# Autodesk Inventor assembly: CH3-chassisFull
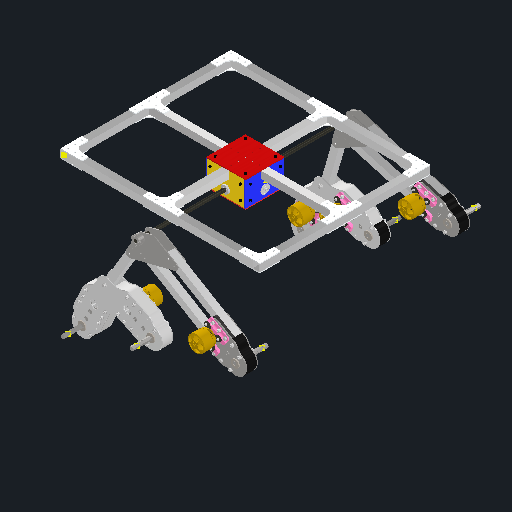
[picture p0: Inventor's stored thumbnail of the model, 512x512]
Saved by Autodesk Inventor 2026.1 (Build 301233020, 233B)
## iProperties
Created: 2025-01-30
Part Number: CH3-chassisFull
Document SubType Name: Assembly
Designer: t205b
Author: t205b
## Documents named in this file (15)
- C:\Users\t205b\OneDrive\Documents\Github\BehrendURCMechanical\CAD\Chassis V3\CH3-chassisFull.iam
- C:\Users\t205b\OneDrive\Documents\Github\BehrendURCMechanical\CAD\Chassis V3\aluminumextrusiontool.ipt
- C:\Users\t205b\OneDrive\Documents\Github\BehrendURCMechanical\CAD\Chassis V3\CH3-L3DoubleGearbox.iam
- C:\Users\t205b\OneDrive\Documents\Github\BehrendURCMechanical\CAD\Chassis V3\CH3-L1SingleGearbox.iam
- C:\Users\t205b\OneDrive\Documents\Github\BehrendURCMechanical\CAD\Chassis V3\HipPivotPlate.ipt
- C:\Users\t205b\OneDrive\Documents\Github\BehrendURCMechanical\CAD\Chassis V3\CH3-PivotBoltNutWasher.iam
- C:\Users\t205b\OneDrive\Documents\Github\BehrendURCMechanical\CAD\Chassis V3\aluminumextrusiontool\aluminumextrusiontool-13.31255in.ipt
- C:\Users\t205b\OneDrive\Documents\Github\BehrendURCMechanical\CAD\Chassis V3\aluminumextrusiontool\aluminumextrusiontool\aluminumextrusiontool-17-13.31255in.ipt
- C:\Users\t205b\OneDrive\Documents\Github\BehrendURCMechanical\CAD\Chassis V3\aluminumextrusiontool\aluminumextrusiontool.ipt
- C:\Users\t205b\OneDrive\Documents\Github\BehrendURCMechanical\CAD\Chassis V3\aluminumextrusiontool\aluminumextrusiontool\aluminumextrusiontool-8in.ipt
- C:\Users\t205b\OneDrive\Documents\Github\BehrendURCMechanical\CAD\Chassis V3\aluminumextrusiontool\aluminumextrusiontool\aluminumextrusiontool-11in.ipt
- C:\Users\t205b\OneDrive\Documents\Github\BehrendURCMechanical\CAD\Chassis V3\Body\CH3-BodyAssembly.iam
- C:\Users\t205b\OneDrive\Documents\Github\BehrendURCMechanical\CAD\Chassis V3\Differential Box\CH3-DiffHousingAsm.iam
- C:\Users\t205b\OneDrive\Documents\Github\BehrendURCMechanical\CAD\Chassis V3\HipCoupler.ipt
- C:\Users\t205b\OneDrive\Documents\Github\BehrendURCMechanical\CAD\Chassis V3\HipCoupler V2.ipt
## Components (22 placed, 12 different names)
1. aluminumextrusiontool-17-13.5in:11 — Mate:31, Mate:32, Mate:33, Mate:38
2. aluminumextrusiontool-8in:12 — Mate:9, Mate:10, Mate:15, Mate:16, Mate:17, Mate:18, Mate:19, Mate:20
3. CH3-L3DoubleGearbox:1 [sub-assembly] — Mate:29, Mate:30
4. CH3-L3DoubleGearbox:2 [sub-assembly] — Mate:4, Mate:5, Mate:22
5. CH3-L1SingleGearbox:1 [sub-assembly] — Mate:37, Mate:38, Mate:39
6. CH3-L1SingleGearbox:2 [sub-assembly] — Mate:46, Mate:47, Mate:48
7. HipPivotPlate:1 — Mate:10, Mate:19, Mate:20, Mate:54, Mate:58, Mate:60
8. HipPivotPlate:2 — Mate:26, Mate:27, Mate:28, Mate:40, Mate:41, Mate:43, Mate:44, Mate:62, Mate:63
9. CH3-PivotBoltNutWasher:1 [sub-assembly] — Mate:9, Mate:16, Mate:29, Mate:30
10. CH3-PivotBoltNutWasher:2 [sub-assembly] — Mate:4, Mate:5, Mate:21
11. HipPivotPlate:3 — Mate:15, Mate:17, Mate:18, Mate:31, Mate:32, Mate:33, Mate:34, Mate:35, Mate:36, Mate:56, Mate:57
12. aluminumextrusiontool-11in:13 — Mate:43, Mate:44, Mate:45, Mate:46
13. aluminumextrusiontool-11in:14 — Mate:34, Mate:35, Mate:36, Mate:37, Mate:39
14. aluminumextrusiontool-13.31255in:10 — Mate:40, Mate:41, Mate:42, Mate:47, Mate:48
15. aluminumextrusiontool-8in:15 — Mate:21, Mate:22, Mate:23, Mate:24, Mate:25, Mate:26, Mate:27, Mate:28
16. HipPivotPlate:4 — Mate:23, Mate:24, Mate:25, Mate:42, Mate:45, Mate:53, Mate:64, Mate:65, Mate:66
17. CH3-BodyAssembly:1 [sub-assembly] — Mate:49, Mate:50, Mate:51, Mate:52
18. Ch3-DiffHousingAsm:1 [sub-assembly] — Mate:49, Mate:50, Mate:51, Mate:52, Mate:53, Mate:54, Mate:55, Mate:59, Mate:61, Flush:1, Flush:2
19. HipCoupler:1 — Mate:58, Mate:59, Mate:60
20. HipCoupler V2:1 — Mate:55, Mate:56, Mate:57, Flush:1
21. HipCoupler:2 — Mate:61, Mate:62, Mate:63
22. HipCoupler V2:2 — Mate:64, Mate:65, Mate:66, Flush:2
## Relationships (58: Mate 56, Flush 2)
- Mate:4: CH3-L3DoubleGearbox:2 ↔ CH3-PivotBoltNutWasher:2
- Mate:5: CH3-L3DoubleGearbox:2 ↔ CH3-PivotBoltNutWasher:2
- Mate:9: aluminumextrusiontool-8in:12 ↔ CH3-PivotBoltNutWasher:1
- Mate:10: aluminumextrusiontool-8in:12 ↔ HipPivotPlate:1
- Mate:15: aluminumextrusiontool-8in:12 ↔ HipPivotPlate:3
- Mate:16: aluminumextrusiontool-8in:12 ↔ CH3-PivotBoltNutWasher:1
- Mate:17: aluminumextrusiontool-8in:12 ↔ HipPivotPlate:3
- Mate:18: aluminumextrusiontool-8in:12 ↔ HipPivotPlate:3
- Mate:19: aluminumextrusiontool-8in:12 ↔ HipPivotPlate:1
- Mate:20: aluminumextrusiontool-8in:12 ↔ HipPivotPlate:1
- Mate:21: CH3-PivotBoltNutWasher:2 ↔ aluminumextrusiontool-8in:15
- Mate:22: CH3-L3DoubleGearbox:2 ↔ aluminumextrusiontool-8in:15
- Mate:23: aluminumextrusiontool-8in:15 ↔ HipPivotPlate:4
- Mate:24: aluminumextrusiontool-8in:15 ↔ HipPivotPlate:4
- Mate:25: aluminumextrusiontool-8in:15 ↔ HipPivotPlate:4
- Mate:26: HipPivotPlate:2 ↔ aluminumextrusiontool-8in:15
- Mate:27: HipPivotPlate:2 ↔ aluminumextrusiontool-8in:15
- Mate:28: HipPivotPlate:2 ↔ aluminumextrusiontool-8in:15
- Mate:29: CH3-L3DoubleGearbox:1 ↔ CH3-PivotBoltNutWasher:1
- Mate:30: CH3-L3DoubleGearbox:1 ↔ CH3-PivotBoltNutWasher:1
- Mate:31: aluminumextrusiontool-17-13.5in:11 ↔ HipPivotPlate:3
- Mate:32: aluminumextrusiontool-17-13.5in:11 ↔ HipPivotPlate:3
- Mate:33: aluminumextrusiontool-17-13.5in:11 ↔ HipPivotPlate:3
- Mate:34: HipPivotPlate:3 ↔ aluminumextrusiontool-11in:14
- Mate:35: HipPivotPlate:3 ↔ aluminumextrusiontool-11in:14
- Mate:36: HipPivotPlate:3 ↔ aluminumextrusiontool-11in:14
- Mate:37: CH3-L1SingleGearbox:1 ↔ aluminumextrusiontool-11in:14
- Mate:38: aluminumextrusiontool-17-13.5in:11 ↔ CH3-L1SingleGearbox:1
- Mate:39: CH3-L1SingleGearbox:1 ↔ aluminumextrusiontool-11in:14
- Mate:40: HipPivotPlate:2 ↔ aluminumextrusiontool-13.31255in:10
- Mate:41: HipPivotPlate:2 ↔ aluminumextrusiontool-13.31255in:10
- Mate:42: aluminumextrusiontool-13.31255in:10 ↔ HipPivotPlate:4
- Mate:43: HipPivotPlate:2 ↔ aluminumextrusiontool-11in:13
- Mate:44: HipPivotPlate:2 ↔ aluminumextrusiontool-11in:13
- Mate:45: aluminumextrusiontool-11in:13 ↔ HipPivotPlate:4
- Mate:46: CH3-L1SingleGearbox:2 ↔ aluminumextrusiontool-11in:13
- Mate:47: CH3-L1SingleGearbox:2 ↔ aluminumextrusiontool-13.31255in:10
- Mate:48: CH3-L1SingleGearbox:2 ↔ aluminumextrusiontool-13.31255in:10
- Mate:49: CH3-BodyAssembly:1 ↔ Ch3-DiffHousingAsm:1
- Mate:50: CH3-BodyAssembly:1 ↔ Ch3-DiffHousingAsm:1
- Mate:51: CH3-BodyAssembly:1 ↔ Ch3-DiffHousingAsm:1
- Mate:52: CH3-BodyAssembly:1 ↔ Ch3-DiffHousingAsm:1
- Mate:53: HipPivotPlate:4 ↔ Ch3-DiffHousingAsm:1
- Mate:54: HipPivotPlate:1 ↔ Ch3-DiffHousingAsm:1
- Mate:55: Ch3-DiffHousingAsm:1 ↔ HipCoupler V2:1
- Mate:56: HipPivotPlate:3 ↔ HipCoupler V2:1
- Mate:57: HipPivotPlate:3 ↔ HipCoupler V2:1
- Mate:58: HipPivotPlate:1 ↔ HipCoupler:1
- Mate:59: Ch3-DiffHousingAsm:1 ↔ HipCoupler:1
- Mate:60: HipPivotPlate:1 ↔ HipCoupler:1
- Mate:61: Ch3-DiffHousingAsm:1 ↔ HipCoupler:2
- Mate:62: HipPivotPlate:2 ↔ HipCoupler:2
- Mate:63: HipPivotPlate:2 ↔ HipCoupler:2
- Mate:64: HipPivotPlate:4 ↔ HipCoupler V2:2
- Mate:65: HipPivotPlate:4 ↔ HipCoupler V2:2
- Mate:66: HipPivotPlate:4 ↔ HipCoupler V2:2
- Flush:1: Ch3-DiffHousingAsm:1 ↔ HipCoupler V2:1
- Flush:2: Ch3-DiffHousingAsm:1 ↔ HipCoupler V2:2
